# Autodesk Inventor assembly: POM_T5_12
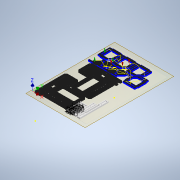
[picture p0: Inventor's stored thumbnail of the model, 180x180]
Saved by Autodesk Inventor 2020 (Build 240168000, 168)
## iProperties
Created: 2021-08-27
Part Number: POM_T5_12
Document SubType Name: Assembly
Designer: Masato
Author: Masato
## Documents named in this file (11)
- C:\Users\L20C1118 森　圭汰\Documents\220428_open\SUSTAINA-OP\Cam\POM_T5_12.iam
- C:\Users\L20C1118 森　圭汰\Documents\220428_open\SUSTAINA-OP\Cam\DisposableBoard.ipt
- C:\Users\L20C1118 森　圭汰\Documents\220428_open\SUSTAINA-OP\UpperBody\Cockpit\Cockpit_side_frame.ipt
- C:\Users\L20C1118 森　圭汰\Documents\220428_open\SUSTAINA-OP\UpperBody\Cockpit\Cockpit_side_frame_MIR.ipt
- C:\Users\L20C1118 森　圭汰\Documents\220428_open\SUSTAINA-OP\Jig\Cockpit_battery_front_frame_Jig.ipt
- C:\Users\L20C1118 森　圭汰\Documents\220428_open\SUSTAINA-OP\Jig\Cockpit_battery_front_frame_Jig_2.ipt
- C:\Users\L20C1118 森　圭汰\Documents\220428_open\SUSTAINA-OP\Jig\Cockpit_carrier_board_frame_Jig.ipt
- C:\Users\L20C1118 森　圭汰\Documents\220428_open\SUSTAINA-OP\Jig\Cockpit_front_frame_Jig.ipt
- C:\Users\L20C1118 森　圭汰\Documents\220428_open\SUSTAINA-OP\Jig\Cockpit_side_frame_Jig.ipt
- C:\Users\L20C1118 森　圭汰\Documents\220428_open\SUSTAINA-OP\UpperBody\Head\Camera_side_frame.ipt
- C:\Users\L20C1118 森　圭汰\Documents\220428_open\SUSTAINA-OP\UpperBody\Arm\ForeArm_diagonal.ipt
## Components (16 placed, 10 different names)
1. DisposableBoard:1 — メイト:2, メイト:1, フラッシュ:1, フラッシュ:2, メイト:4, フラッシュ:3, フラッシュ:4, メイト:7, メイト:8, メイト:9, メイト:10, メイト:11, メイト:17, メイト:22, メイト:23, メイト:24, メイト:25, メイト:29, メイト:31, メイト:32, メイト:36
2. Cockpit_side_frame:1 — メイト:4, フラッシュ:3, フラッシュ:4, フラッシュ:5, メイト:12, メイト:18, メイト:19, フラッシュ:10
3. Cockpit_side_frame_MIR:1 — メイト:17, メイト:18, メイト:19, メイト:26, メイト:38
4. Cockpit_battery_front_frame_Jig:1 — メイト:7, フラッシュ:6, フラッシュ:7, メイト:16, メイト:20, メイト:21
5. Cockpit_battery_front_frame_Jig_2:1 — メイト:8, フラッシュ:5, メイト:12, フラッシュ:6, フラッシュ:9, メイト:20
6. Cockpit_carrier_board_frame_Jig:1 — メイト:9, フラッシュ:8, メイト:15
7. Cockpit_front_frame_Jig:1 — メイト:10, フラッシュ:7, フラッシュ:8, メイト:15, メイト:21
8. Cockpit_side_frame_Jig:1 — メイト:11, メイト:16, フラッシュ:9
9. Camera_side_frame:1 — メイト:22, フラッシュ:10, メイト:26, 正接:1, 正接:2, メイト:27, フラッシュ:11, フラッシュ:13
10. Camera_side_frame:2 — メイト:23, 正接:1, 正接:2, フラッシュ:12, メイト:28, メイト:33
11. Camera_side_frame:3 — メイト:24, メイト:27, フラッシュ:11
12. Camera_side_frame:4 — メイト:25, フラッシュ:12, メイト:28, メイト:39
13. ForeArm_diagonal:1 — メイト:32, フラッシュ:14, メイト:34, フラッシュ:15, メイト:35
14. ForeArm_diagonal:2 — メイト:31, フラッシュ:15, メイト:35
15. ForeArm_diagonal:4 — メイト:29, フラッシュ:13, メイト:33, フラッシュ:14, メイト:34
16. ForeArm_diagonal:5 — メイト:36, メイト:38, メイト:39
## Relationships (49: Mate 32, Flush 15, Tangent 2)
- メイト:2 [Mate]: DisposableBoard:1
- メイト:1 [Mate]: DisposableBoard:1
- フラッシュ:1 [Flush]: DisposableBoard:1
- フラッシュ:2 [Flush]: DisposableBoard:1
- メイト:4 [Mate]: DisposableBoard:1 ↔ Cockpit_side_frame:1
- フラッシュ:3 [Flush] (2.5 mm): DisposableBoard:1 ↔ Cockpit_side_frame:1
- フラッシュ:4 [Flush] (-2.5 mm): DisposableBoard:1 ↔ Cockpit_side_frame:1
- メイト:7 [Mate]: DisposableBoard:1 ↔ Cockpit_battery_front_frame_Jig:1
- メイト:8 [Mate]: DisposableBoard:1 ↔ Cockpit_battery_front_frame_Jig_2:1
- メイト:9 [Mate]: DisposableBoard:1 ↔ Cockpit_carrier_board_frame_Jig:1
- メイト:10 [Mate]: DisposableBoard:1 ↔ Cockpit_front_frame_Jig:1
- メイト:11 [Mate]: DisposableBoard:1 ↔ Cockpit_side_frame_Jig:1
- フラッシュ:5 [Flush]: Cockpit_side_frame:1 ↔ Cockpit_battery_front_frame_Jig_2:1
- メイト:12 [Mate] (2.5 mm): Cockpit_side_frame:1 ↔ Cockpit_battery_front_frame_Jig_2:1
- フラッシュ:6 [Flush]: Cockpit_battery_front_frame_Jig:1 ↔ Cockpit_battery_front_frame_Jig_2:1
- フラッシュ:7 [Flush]: Cockpit_battery_front_frame_Jig:1 ↔ Cockpit_front_frame_Jig:1
- フラッシュ:8 [Flush]: Cockpit_carrier_board_frame_Jig:1 ↔ Cockpit_front_frame_Jig:1
- メイト:15 [Mate] (2.5 mm): Cockpit_carrier_board_frame_Jig:1 ↔ Cockpit_front_frame_Jig:1
- メイト:16 [Mate] (2.5 mm): Cockpit_battery_front_frame_Jig:1 ↔ Cockpit_side_frame_Jig:1
- フラッシュ:9 [Flush]: Cockpit_battery_front_frame_Jig_2:1 ↔ Cockpit_side_frame_Jig:1
- メイト:17 [Mate]: DisposableBoard:1 ↔ Cockpit_side_frame_MIR:1
- メイト:18 [Mate] (2.5 mm): Cockpit_side_frame:1 ↔ Cockpit_side_frame_MIR:1
- メイト:19 [Mate] (2.5 mm): Cockpit_side_frame:1 ↔ Cockpit_side_frame_MIR:1
- メイト:20 [Mate] (2.5 mm): Cockpit_battery_front_frame_Jig:1 ↔ Cockpit_battery_front_frame_Jig_2:1
- メイト:21 [Mate] (2.5 mm): Cockpit_battery_front_frame_Jig:1 ↔ Cockpit_front_frame_Jig:1
- メイト:22 [Mate]: DisposableBoard:1 ↔ Camera_side_frame:1
- メイト:23 [Mate]: DisposableBoard:1 ↔ Camera_side_frame:2
- メイト:24 [Mate]: DisposableBoard:1 ↔ Camera_side_frame:3
- メイト:25 [Mate]: DisposableBoard:1 ↔ Camera_side_frame:4
- フラッシュ:10 [Flush]: Cockpit_side_frame:1 ↔ Camera_side_frame:1
- メイト:26 [Mate] (2.5 mm): Cockpit_side_frame_MIR:1 ↔ Camera_side_frame:1
- 正接:1 [Tangent] (2.5 mm): Camera_side_frame:1 ↔ Camera_side_frame:2
- 正接:2 [Tangent] (2.5 mm): Camera_side_frame:1 ↔ Camera_side_frame:2
- メイト:27 [Mate] (2.5 mm): Camera_side_frame:1 ↔ Camera_side_frame:3
- フラッシュ:11 [Flush]: Camera_side_frame:1 ↔ Camera_side_frame:3
- フラッシュ:12 [Flush]: Camera_side_frame:2 ↔ Camera_side_frame:4
- メイト:28 [Mate] (2.5 mm): Camera_side_frame:2 ↔ Camera_side_frame:4
- メイト:29 [Mate]: DisposableBoard:1 ↔ ForeArm_diagonal:4
- メイト:31 [Mate]: DisposableBoard:1 ↔ ForeArm_diagonal:2
- メイト:32 [Mate]: DisposableBoard:1 ↔ ForeArm_diagonal:1
- フラッシュ:13 [Flush]: Camera_side_frame:1 ↔ ForeArm_diagonal:4
- メイト:33 [Mate] (2.5 mm): Camera_side_frame:2 ↔ ForeArm_diagonal:4
- フラッシュ:14 [Flush]: ForeArm_diagonal:1 ↔ ForeArm_diagonal:4
- メイト:34 [Mate] (2.5 mm): ForeArm_diagonal:1 ↔ ForeArm_diagonal:4
- フラッシュ:15 [Flush]: ForeArm_diagonal:1 ↔ ForeArm_diagonal:2
- メイト:35 [Mate] (2.5 mm): ForeArm_diagonal:1 ↔ ForeArm_diagonal:2
- メイト:36 [Mate]: DisposableBoard:1 ↔ ForeArm_diagonal:5
- メイト:38 [Mate]: Cockpit_side_frame_MIR:1 ↔ ForeArm_diagonal:5
- メイト:39 [Mate] (2.5 mm): Camera_side_frame:4 ↔ ForeArm_diagonal:5
